# Autodesk Inventor assembly: GearSensorCase
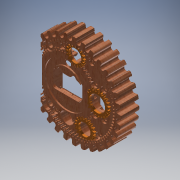
[picture p0: Inventor's stored thumbnail of the model, 180x180]
Saved by Autodesk Inventor 2017 (Build 210142000, 142)
## iProperties
Created: 2017-02-14
Part Number: GearSensorCase
Document SubType Name: Assembly
Designer: Moonlight.Admin
Author: Moonlight.Admin
## Documents named in this file (8)
- E:\FRC\SteamWorks\GearSensorCase.iam
- E:\FRC\SteamWorks\GearSensorCase.ipt
- E:\FRC\SteamWorks\UltrasonicClamp.ipt
- E:\FRC\SteamWorks\IRClamp.ipt
- E:\FRC\SteamWorks\IRGear.ipt
- E:\FRC\SteamWorks\CreeGear.ipt
- E:\FRC\SteamWorks\UltrasonicGear.ipt
- E:\FRC\SteamWorks\LifeCamBot.ipt
## Components (7 placed, 7 different names)
1. GearSensorCase:1 — Mate:1, Mate:2, Mate:4, Mate:5, Mate:6, Mate:7, Mate:8, Mate:9, Mate:10, Mate:11, Mate:13, Mate:14, Mate:15, Mate:16, Mate:17
2. UltrasonicClamp:1 — Mate:1, Mate:2, Mate:17
3. IRClamp:1 — Mate:4, Mate:5, Mate:6
4. IRGear:1 — Mate:7, Mate:8
5. CreeGear:1 — Mate:9, Mate:10
6. UltrasonicGear:1 — Mate:11, Mate:13
7. LifeCamBot:1 — Mate:14, Mate:15, Mate:16
## Relationships (15: Mate 15)
- Mate:1: GearSensorCase:1 ↔ UltrasonicClamp:1
- Mate:2: GearSensorCase:1 ↔ UltrasonicClamp:1
- Mate:4: GearSensorCase:1 ↔ IRClamp:1
- Mate:5: GearSensorCase:1 ↔ IRClamp:1
- Mate:6: GearSensorCase:1 ↔ IRClamp:1
- Mate:7: GearSensorCase:1 ↔ IRGear:1
- Mate:8: GearSensorCase:1 ↔ IRGear:1
- Mate:9: GearSensorCase:1 ↔ CreeGear:1
- Mate:10: GearSensorCase:1 ↔ CreeGear:1
- Mate:11: GearSensorCase:1 ↔ UltrasonicGear:1
- Mate:13: GearSensorCase:1 ↔ UltrasonicGear:1
- Mate:14: GearSensorCase:1 ↔ LifeCamBot:1
- Mate:15: GearSensorCase:1 ↔ LifeCamBot:1
- Mate:16: GearSensorCase:1 ↔ LifeCamBot:1
- Mate:17: GearSensorCase:1 ↔ UltrasonicClamp:1
